# Autodesk Inventor assembly: still pipe
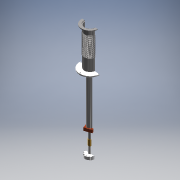
[picture p0: Inventor's stored thumbnail of the model, 180x180]
Saved by Autodesk Inventor 2018 (Build 220112000, 112)
## iProperties
Created: 2019-01-14
Part Number: still pipe
Document SubType Name: Assembly
Designer: Admin
Author: Admin
## Documents named in this file (9)
- C:\Users\Admin\Documents\Cryostat\CAD\still pipe.iam
- C:\Users\Admin\Documents\Cryostat\CAD\KF50 bellows.ipt
- C:\Users\Admin\Documents\Cryostat\CAD\universal connector.ipt
- C:\Users\Admin\Documents\Cryostat\CAD\silverSolderJoint.ipt
- C:\Users\Admin\Documents\Cryostat\CAD\1in ss pipe.ipt
- C:\Users\Admin\Documents\Cryostat\CAD\0in5 ss pipe.ipt
- C:\Users\Admin\Documents\Cryostat\CAD\brassbushing.ipt
- C:\Users\Admin\Documents\Cryostat\CAD\adapter.ipt
- C:\Users\Admin\Documents\Cryostat\CAD\heatsink.ipt
## Components (8 placed, 8 different names)
1. KF50 bellows:1 — Mate:16, Flush:2
2. universal connector:1 — Mate:12, Mate:13
3. silverSolderJoint:1 — Mate:6, Mate:8, Mate:9, Mate:10
4. 1in ss pipe:3 — Mate:6, Mate:8, Mate:15, Flush:1, Mate:17
5. 0in5 ss pipe:1 — Mate:9, Mate:10, Mate:11, Mate:13, Mate:14
6. brassbushing:1 — Mate:11, Mate:12, Mate:14
7. adapter:1 — Mate:15, Flush:1, Mate:16, Flush:2, Mate:18, Mate:19
8. heatsink:1 — Mate:17, Mate:18, Mate:19
## Relationships (15: Mate 13, Flush 2)
- Mate:6: silverSolderJoint:1 ↔ 1in ss pipe:3
- Mate:8: silverSolderJoint:1 ↔ 1in ss pipe:3
- Mate:9: silverSolderJoint:1 ↔ 0in5 ss pipe:1
- Mate:10: silverSolderJoint:1 ↔ 0in5 ss pipe:1
- Mate:11: 0in5 ss pipe:1 ↔ brassbushing:1
- Mate:12: universal connector:1 ↔ brassbushing:1
- Mate:13 (5.08 mm): universal connector:1 ↔ 0in5 ss pipe:1
- Mate:14 (-10.16 mm): 0in5 ss pipe:1 ↔ brassbushing:1
- Mate:15: 1in ss pipe:3 ↔ adapter:1
- Flush:1: 1in ss pipe:3 ↔ adapter:1
- Mate:16: KF50 bellows:1 ↔ adapter:1
- Flush:2: KF50 bellows:1 ↔ adapter:1
- Mate:17: 1in ss pipe:3 ↔ heatsink:1
- Mate:18: adapter:1 ↔ heatsink:1
- Mate:19: adapter:1 ↔ heatsink:1
